# Autodesk Inventor assembly: Main
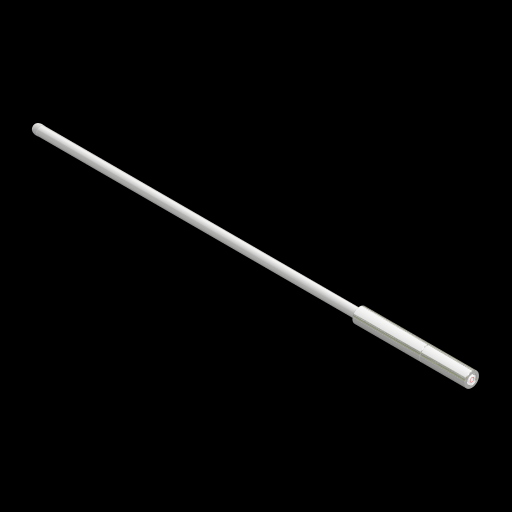
[picture p0: Inventor's stored thumbnail of the model, 512x512]
Saved by Autodesk Inventor 2023 (Build 270158000, 158)
## iProperties
Created: 2022-02-04
Part Number: Main
Document SubType Name: Assembly
Designer: Michael Lacey
Mass: 1181.48 g
Surface Area: 4169 cm^2
Volume: 721.445 cm^3
Density: 1.63766 g/cm^3
Author: Michael Lacey
## Documents named in this file (5)
- C:\Users\foams\3D Objects\Light Saber\All Files Compiled\CAD\Main.iam
- C:\Users\foams\3D Objects\Light Saber\All Files Compiled\CAD\ProtoModelMake.iam
- C:\Users\foams\3D Objects\Light Saber\All Files Compiled\CAD\Assembly1.iam
- C:\Users\foams\3D Objects\Light Saber\All Files Compiled\CAD\BatteryHousing.iam
- C:\Users\foams\3D Objects\Light Saber\All Files Compiled\CAD\Blade Assembly.iam
## Components (4 placed, 4 different names)
1. ProtoModelMake:1 [sub-assembly] — Mate:4, Mate:8, Mate:12, Mate:13, Flush:1
2. Assembly1:1 [sub-assembly] — Mate:4, Flush:1
3. BatteryHousing:1 [sub-assembly] — Mate:8
4. Blade Assembly:1 [sub-assembly] — Mate:12, Mate:13
## Relationships (5: Mate 4, Flush 1)
- Mate:4: ProtoModelMake:1 ↔ Assembly1:1
- Mate:8: ProtoModelMake:1 ↔ BatteryHousing:1
- Mate:12: ProtoModelMake:1 ↔ Blade Assembly:1
- Mate:13: ProtoModelMake:1 ↔ Blade Assembly:1
- Flush:1: ProtoModelMake:1 ↔ Assembly1:1
